# Autodesk Inventor assembly: ASY PNS 1750 filter-distribution-system 1200_1600
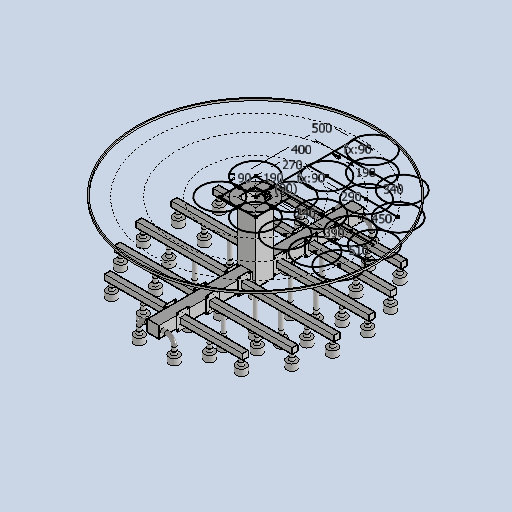
[picture p0: Inventor's stored thumbnail of the model, 512x512]
Saved by Autodesk Inventor 2025.1 (Build 291241020, 241B)
## iProperties
Created: 2025-06-24
Part Number: ASY PNS 1750 filter-distribution-system 1200_1600
Document SubType Name: Assembly
Designer: admin
Author: user
## Documents named in this file (14)
- C:\Users\user\YandexDisk-badmisterfox\home pc\Inventor\PNS2-Panaevsk\Filter D1000\filter-distribution-system 1000\ASY PNS 1750 filter-distribution-system 1200_1600.iam
- C:\Users\user\YandexDisk-badmisterfox\home pc\Inventor\PNS2-Panaevsk\Filter D1000\filter-distribution-system 1000\PNS 1759 DIM filter-distribution-system 1200_1600.ipt
- C:\Users\user\YandexDisk-badmisterfox\home pc\Inventor\PNS2-Panaevsk\Filter D1000\filter-distribution-system 1000\PNS 754 FDS 1200 FLANGE_1600.ipt
- C:\Users\user\YandexDisk-badmisterfox\home pc\Inventor\PNS2-Panaevsk\Filter D1000\filter-distribution-system 1000\PNS 752 FDS 1200 FLANGE 2_1600.ipt
- C:\Users\user\YandexDisk-badmisterfox\home pc\Inventor\PNS2-Panaevsk\Filter D1000\filter-distribution-system 1000\PNS 753 FDS 1200 FLANGE 3_1600.ipt
- C:\Users\user\YandexDisk-badmisterfox\home pc\Inventor\PNS2-Panaevsk\CC\en-US\JIS B 2312 90 (4)\JIS B 2312 90 Deg Long Elbow Stainless Steel 15A x Sch 5S.ipt
- C:\Users\user\YandexDisk-badmisterfox\home pc\Inventor\PNS2-Panaevsk\Filter D1000\filter-distribution-system 1000\PNS dummy filter element_1600.ipt
- C:\Users\user\YandexDisk-badmisterfox\home pc\Inventor\PNS2-Panaevsk\Filter D1000\filter-distribution-system 1000\PNS dummy pipe nippel_1600.ipt
- C:\Users\user\YandexDisk-badmisterfox\home pc\Inventor\PNS2-Panaevsk\Filter D1000\filter-distribution-system 1000\ASY PNS FDS way1_1600.iam
- C:\Users\user\YandexDisk-badmisterfox\home pc\Inventor\PNS2-Panaevsk\Filter D1000\filter-distribution-system 1000\ASY PNS 1752 FDS way 2_1600.iam
- C:\Users\user\YandexDisk-badmisterfox\home pc\Inventor\PNS2-Panaevsk\Filter D1000\filter-distribution-system 1000\ASY PNS FDS way3_1600.iam
- C:\Users\user\YandexDisk-badmisterfox\home pc\Inventor\PNS2-Panaevsk\Filter D1000\filter-distribution-system 1000\PNS 1757 FDS 1200 way tube 7_1600.ipt
- C:\Users\user\YandexDisk-badmisterfox\home pc\Inventor\PNS2-Panaevsk\Filter D1000\filter-distribution-system 1000\PNS 767 FDS 1200 CUP 2_1600.ipt
- C:\Users\user\YandexDisk-badmisterfox\home pc\Inventor\PNS2-Panaevsk\Filter D1000\filter-distribution-system 1000\PNS 765 FDS 1200 CUP 1_1600.ipt
## Components (37 placed, 13 different names)
1. PNS 1759 DIM filter-distribution-system 1200_1600:1 — Mate:5, Mate:4
2. PNS 754 FDS 1200 FLANGE_1600:1 — Flush:1, Flush:2, Mate:1
3. PNS 752 FDS 1200 FLANGE 2_1600:1 — Flush:1, Flush:4, Flush:3, Mate:6, Rigid:1, Rigid:2
4. PNS 752 FDS 1200 FLANGE 2_1600:2 — Flush:2, Mate:1, Rigid:1, Rigid:3
5. PNS 753 FDS 1200 FLANGE 3_1600:1 — Rigid:2, Rigid:7, Rigid:4, Rigid:5, Rigid:6, Rigid:9, Rigid:14, Rigid:15, Rigid:31, Rigid:33
6. PNS 753 FDS 1200 FLANGE 3_1600:2 — Rigid:3, Rigid:11, Rigid:10, Rigid:13, Rigid:12, Rigid:16, Rigid:17, Rigid:29, Rigid:30, Rigid:32
7. JIS B 2312 90 Deg Long Elbow Stainless Steel 15A x Sch 5S:1 — Rigid:7, Rigid:8, Rigid:18, Rigid:19
8. PNS dummy filter element_1600:1 — Rigid:8
9. PNS dummy pipe nippel_1600:1 — Rigid:18
10. ASY PNS FDS way1_1600:1 [sub-assembly] — Rigid:4
11. ASY PNS 1752 FDS way 2_1600:1 [sub-assembly] — Rigid:5
12. ASY PNS FDS way3_1600:1 [sub-assembly] — Rigid:6
13. ASY PNS FDS way1_1600:2 [sub-assembly] — Rigid:9
14. ASY PNS FDS way1_1600:3 [sub-assembly] — Rigid:11
15. ASY PNS FDS way1_1600:4 [sub-assembly] — Rigid:10
16. ASY PNS 1752 FDS way 2_1600:2 [sub-assembly] — Rigid:14
17. ASY PNS 1752 FDS way 2_1600:3 [sub-assembly] — Rigid:13
18. ASY PNS 1752 FDS way 2_1600:4 [sub-assembly] — Rigid:12
19. ASY PNS FDS way3_1600:2 [sub-assembly] — Rigid:15
20. ASY PNS FDS way3_1600:3 [sub-assembly] — Rigid:16
21. ASY PNS FDS way3_1600:4 [sub-assembly] — Rigid:17
22. PNS 1757 FDS 1200 way tube 7_1600:1 — Rigid:19
23. JIS B 2312 90 Deg Long Elbow Stainless Steel 15A x Sch 5S:2 — Rigid:20, Rigid:21, Rigid:22
24. PNS dummy filter element_1600:2 — Rigid:20
25. PNS dummy pipe nippel_1600:2 — Rigid:21
26. PNS 1757 FDS 1200 way tube 7_1600:2 — Rigid:31, Rigid:22
27. JIS B 2312 90 Deg Long Elbow Stainless Steel 15A x Sch 5S:3 — Rigid:23, Rigid:24, Rigid:25
28. PNS dummy filter element_1600:3 — Rigid:23
29. PNS dummy pipe nippel_1600:3 — Rigid:24
30. PNS 1757 FDS 1200 way tube 7_1600:3 — Rigid:29, Rigid:25
31. JIS B 2312 90 Deg Long Elbow Stainless Steel 15A x Sch 5S:4 — Rigid:26, Rigid:27, Rigid:28
32. PNS dummy filter element_1600:4 — Rigid:26
33. PNS dummy pipe nippel_1600:4 — Rigid:27
34. PNS 1757 FDS 1200 way tube 7_1600:4 — Rigid:30, Rigid:28
35. PNS 767 FDS 1200 CUP 2_1600:1 — Rigid:32
36. PNS 767 FDS 1200 CUP 2_1600:2 — Rigid:33
37. PNS 765 FDS 1200 CUP 1_1600:1 — Flush:4, Flush:3, Mate:6
## Relationships (41: WeldJoint 33, Mate 4, Flush 4)
- Mate:5: PNS 1759 DIM filter-distribution-system 1200_1600:1
- Mate:4: PNS 1759 DIM filter-distribution-system 1200_1600:1
- Flush:1: PNS 754 FDS 1200 FLANGE_1600:1 ↔ PNS 752 FDS 1200 FLANGE 2_1600:1
- Flush:2: PNS 754 FDS 1200 FLANGE_1600:1 ↔ PNS 752 FDS 1200 FLANGE 2_1600:2
- Mate:1: PNS 754 FDS 1200 FLANGE_1600:1 ↔ PNS 752 FDS 1200 FLANGE 2_1600:2
- Flush:4: PNS 752 FDS 1200 FLANGE 2_1600:1 ↔ PNS 765 FDS 1200 CUP 1_1600:1
- Flush:3: PNS 752 FDS 1200 FLANGE 2_1600:1 ↔ PNS 765 FDS 1200 CUP 1_1600:1
- Mate:6: PNS 752 FDS 1200 FLANGE 2_1600:1 ↔ PNS 765 FDS 1200 CUP 1_1600:1
- Rigid:1 [WeldJoint]: PNS 752 FDS 1200 FLANGE 2_1600:1 ↔ PNS 752 FDS 1200 FLANGE 2_1600:2
- Rigid:2 [WeldJoint]: PNS 752 FDS 1200 FLANGE 2_1600:1 ↔ PNS 753 FDS 1200 FLANGE 3_1600:1
- Rigid:3 [WeldJoint]: PNS 752 FDS 1200 FLANGE 2_1600:2 ↔ PNS 753 FDS 1200 FLANGE 3_1600:2
- Rigid:7 [WeldJoint] (-20 mm): PNS 753 FDS 1200 FLANGE 3_1600:1 ↔ JIS B 2312 90 Deg Long Elbow Stainless Steel 15A x Sch 5S:1
- Rigid:8 [WeldJoint] (20 mm): JIS B 2312 90 Deg Long Elbow Stainless Steel 15A x Sch 5S:1 ↔ PNS dummy filter element_1600:1
- Rigid:18 [WeldJoint]: JIS B 2312 90 Deg Long Elbow Stainless Steel 15A x Sch 5S:1 ↔ PNS dummy pipe nippel_1600:1
- Rigid:4 [WeldJoint] (-2 mm): PNS 753 FDS 1200 FLANGE 3_1600:1 ↔ ASY PNS FDS way1_1600:1
- Rigid:5 [WeldJoint] (-2 mm): PNS 753 FDS 1200 FLANGE 3_1600:1 ↔ ASY PNS 1752 FDS way 2_1600:1
- Rigid:6 [WeldJoint]: PNS 753 FDS 1200 FLANGE 3_1600:1 ↔ ASY PNS FDS way3_1600:1
- Rigid:9 [WeldJoint]: PNS 753 FDS 1200 FLANGE 3_1600:1 ↔ ASY PNS FDS way1_1600:2
- Rigid:11 [WeldJoint]: PNS 753 FDS 1200 FLANGE 3_1600:2 ↔ ASY PNS FDS way1_1600:3
- Rigid:10 [WeldJoint]: PNS 753 FDS 1200 FLANGE 3_1600:2 ↔ ASY PNS FDS way1_1600:4
- Rigid:14 [WeldJoint]: PNS 753 FDS 1200 FLANGE 3_1600:1 ↔ ASY PNS 1752 FDS way 2_1600:2
- Rigid:13 [WeldJoint]: PNS 753 FDS 1200 FLANGE 3_1600:2 ↔ ASY PNS 1752 FDS way 2_1600:3
- Rigid:12 [WeldJoint]: PNS 753 FDS 1200 FLANGE 3_1600:2 ↔ ASY PNS 1752 FDS way 2_1600:4
- Rigid:15 [WeldJoint]: PNS 753 FDS 1200 FLANGE 3_1600:1 ↔ ASY PNS FDS way3_1600:2
- Rigid:16 [WeldJoint]: PNS 753 FDS 1200 FLANGE 3_1600:2 ↔ ASY PNS FDS way3_1600:3
- Rigid:17 [WeldJoint]: PNS 753 FDS 1200 FLANGE 3_1600:2 ↔ ASY PNS FDS way3_1600:4
- Rigid:19 [WeldJoint]: JIS B 2312 90 Deg Long Elbow Stainless Steel 15A x Sch 5S:1 ↔ PNS 1757 FDS 1200 way tube 7_1600:1
- Rigid:20 [WeldJoint] (20 mm): JIS B 2312 90 Deg Long Elbow Stainless Steel 15A x Sch 5S:2 ↔ PNS dummy filter element_1600:2
- Rigid:21 [WeldJoint]: JIS B 2312 90 Deg Long Elbow Stainless Steel 15A x Sch 5S:2 ↔ PNS dummy pipe nippel_1600:2
- Rigid:31 [WeldJoint]: PNS 753 FDS 1200 FLANGE 3_1600:1 ↔ PNS 1757 FDS 1200 way tube 7_1600:2
- Rigid:22 [WeldJoint]: JIS B 2312 90 Deg Long Elbow Stainless Steel 15A x Sch 5S:2 ↔ PNS 1757 FDS 1200 way tube 7_1600:2
- Rigid:23 [WeldJoint] (20 mm): JIS B 2312 90 Deg Long Elbow Stainless Steel 15A x Sch 5S:3 ↔ PNS dummy filter element_1600:3
- Rigid:24 [WeldJoint]: JIS B 2312 90 Deg Long Elbow Stainless Steel 15A x Sch 5S:3 ↔ PNS dummy pipe nippel_1600:3
- Rigid:29 [WeldJoint]: PNS 753 FDS 1200 FLANGE 3_1600:2 ↔ PNS 1757 FDS 1200 way tube 7_1600:3
- Rigid:25 [WeldJoint]: JIS B 2312 90 Deg Long Elbow Stainless Steel 15A x Sch 5S:3 ↔ PNS 1757 FDS 1200 way tube 7_1600:3
- Rigid:26 [WeldJoint] (20 mm): JIS B 2312 90 Deg Long Elbow Stainless Steel 15A x Sch 5S:4 ↔ PNS dummy filter element_1600:4
- Rigid:27 [WeldJoint]: JIS B 2312 90 Deg Long Elbow Stainless Steel 15A x Sch 5S:4 ↔ PNS dummy pipe nippel_1600:4
- Rigid:30 [WeldJoint]: PNS 753 FDS 1200 FLANGE 3_1600:2 ↔ PNS 1757 FDS 1200 way tube 7_1600:4
- Rigid:28 [WeldJoint]: JIS B 2312 90 Deg Long Elbow Stainless Steel 15A x Sch 5S:4 ↔ PNS 1757 FDS 1200 way tube 7_1600:4
- Rigid:32 [WeldJoint]: PNS 753 FDS 1200 FLANGE 3_1600:2 ↔ PNS 767 FDS 1200 CUP 2_1600:1
- Rigid:33 [WeldJoint]: PNS 753 FDS 1200 FLANGE 3_1600:1 ↔ PNS 767 FDS 1200 CUP 2_1600:2
